# Autodesk Inventor assembly: Frame
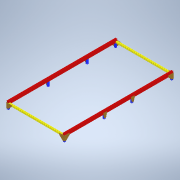
[picture p0: Inventor's stored thumbnail of the model, 180x180]
Saved by Autodesk Inventor 2022.2 (Build 262287010, 287A)
## iProperties
Created: 2022-03-31
Part Number: Frame
Document SubType Name: Assembly
Designer: Robert Nies
Author: Robert Nies
## Documents named in this file (6)
- C:\Users\rober\PycharmProjects\CNCRouter\Master Assembly\Frame.iam
- C:\Users\rober\PycharmProjects\CNCRouter\Master Assembly\Frame Long.ipt
- C:\Users\rober\PycharmProjects\CNCRouter\Master Assembly\Frame Short.ipt
- C:\Users\rober\PycharmProjects\CNCRouter\Master Assembly\Leg.ipt
- C:\Users\rober\PycharmProjects\CNCRouter\Stock Parts\Brackets\90 Deg 5 Hole Bracket.ipt
- C:\Users\rober\PycharmProjects\CNCRouter\Stock Parts\Brackets\Tee 4 Hole Bracket.ipt
## Components (26 placed, 5 different names)
1. Frame Short:2 — Mate:8, Flush:15, Flush:16, Flush:26, Flush:33, Flush:43, Flush:45, Flush:47
2. Frame Short:1 — Mate:3, Flush:5, Flush:6, Flush:13, Mate:7, Flush:14, Flush:20, Flush:39, Flush:41
3. Frame Long:1 — Flush:1, Flush:2, Mate:1, Mate:20, Flush:32, Mate:21, Flush:34, Mate:22, Flush:35, Mate:29, Flush:48
4. Frame Long:2 — Flush:1, Flush:2, Mate:1, Mate:3, Flush:5, Flush:6, Flush:17, Mate:9, Flush:18, Mate:19, Flush:31, Mate:23, Flush:36, Mate:25, Mate:26
5. Frame Long:3 — Flush:3, Flush:4, Mate:2, Mate:8, Flush:15, Flush:16, Flush:24, Mate:14, Mate:15, Mate:17, Flush:27, Flush:28, Flush:29, Mate:18, Mate:27, Mate:28, Flush:46
6. Frame Long:4 — Flush:3, Flush:4, Mate:2, Mate:6, Flush:11, Flush:12, Flush:13, Mate:7, Flush:14, Flush:19, Mate:11, Mate:12, Flush:23
7. Leg:8 — Mate:23, Flush:36, Mate:24
8. Leg:7 — Mate:21, Flush:33, Flush:34, Mate:30, Flush:50
9. Leg:6 — Mate:15, Mate:16, Flush:26, Flush:27, Flush:44
10. Leg:5 — Mate:10, Flush:19, Mate:11, Flush:25
11. Leg:4 — Mate:16, Mate:17, Flush:28, Flush:30
12. Leg:3 — Mate:22, Flush:35, Flush:38
13. Leg:2 — Flush:17, Mate:9, Flush:18, Mate:24, Flush:40
14. Leg:1 — Mate:6, Flush:11, Flush:12, Mate:10, Flush:21, Mate:13
15. 90 Deg 5 Hole Bracket:3 — Mate:25, Flush:39, Flush:40, Flush:42
16. 90 Deg 5 Hole Bracket:4 — Mate:26, Flush:41, Flush:42
17. 90 Deg 5 Hole Bracket:5 — Mate:27, Flush:43, Flush:44
18. 90 Deg 5 Hole Bracket:6 — Mate:28, Flush:45, Flush:46
19. 90 Deg 5 Hole Bracket:7 — Flush:47, Mate:29, Flush:48, Flush:49
20. 90 Deg 5 Hole Bracket:8 — Mate:30, Flush:49, Flush:50
21. Tee 4 Hole Bracket:2 — Flush:29, Mate:18, Flush:30
22. Tee 4 Hole Bracket:3 — Mate:19, Flush:31, Flush:37
23. Tee 4 Hole Bracket:4 — Mate:20, Flush:32, Flush:38
24. Tee 4 Hole Bracket:1 — Flush:24, Mate:14, Flush:25, Flush:37
25. 90 Deg 5 Hole Bracket:2 — Flush:22, Mate:13, Flush:23
26. 90 Deg 5 Hole Bracket:1 — Flush:20, Flush:21, Mate:12, Flush:22
## Relationships (74: Flush 46, Mate 28)
- Flush:1: Frame Long:1 ↔ Frame Long:2
- Flush:2: Frame Long:1 ↔ Frame Long:2
- Mate:1: Frame Long:1 ↔ Frame Long:2
- Flush:3: Frame Long:3 ↔ Frame Long:4
- Flush:4: Frame Long:3 ↔ Frame Long:4
- Mate:2: Frame Long:3 ↔ Frame Long:4
- Mate:3: Frame Short:1 ↔ Frame Long:2
- Flush:5: Frame Short:1 ↔ Frame Long:2
- Flush:6: Frame Short:1 ↔ Frame Long:2
- Mate:6: Frame Long:4 ↔ Leg:1
- Flush:11: Frame Long:4 ↔ Leg:1
- Flush:12: Frame Long:4 ↔ Leg:1
- Flush:13: Frame Short:1 ↔ Frame Long:4
- Mate:7: Frame Short:1 ↔ Frame Long:4
- Flush:14: Frame Short:1 ↔ Frame Long:4
- Mate:8: Frame Short:2 ↔ Frame Long:3
- Flush:15: Frame Short:2 ↔ Frame Long:3
- Flush:16: Frame Short:2 ↔ Frame Long:3
- Flush:17: Frame Long:2 ↔ Leg:2
- Mate:9: Frame Long:2 ↔ Leg:2
- Flush:18: Frame Long:2 ↔ Leg:2
- Mate:10 (889 mm): Leg:5 ↔ Leg:1
- Flush:19: Frame Long:4 ↔ Leg:5
- Mate:11: Frame Long:4 ↔ Leg:5
- Flush:20: Frame Short:1 ↔ 90 Deg 5 Hole Bracket:1
- Flush:21: Leg:1 ↔ 90 Deg 5 Hole Bracket:1
- Mate:12: Frame Long:4 ↔ 90 Deg 5 Hole Bracket:1
- Flush:22: 90 Deg 5 Hole Bracket:2 ↔ 90 Deg 5 Hole Bracket:1
- Mate:13: Leg:1 ↔ 90 Deg 5 Hole Bracket:2
- Flush:23: Frame Long:4 ↔ 90 Deg 5 Hole Bracket:2
- Flush:24 (38.1 mm): Frame Long:3 ↔ Tee 4 Hole Bracket:1
- Mate:14: Frame Long:3 ↔ Tee 4 Hole Bracket:1
- Flush:25 (19.05 mm): Leg:5 ↔ Tee 4 Hole Bracket:1
- Mate:15: Frame Long:3 ↔ Leg:6
- Mate:16 (889 mm): Leg:6 ↔ Leg:4
- Mate:17: Frame Long:3 ↔ Leg:4
- Flush:26: Frame Short:2 ↔ Leg:6
- Flush:27: Frame Long:3 ↔ Leg:6
- Flush:28: Frame Long:3 ↔ Leg:4
- Flush:29 (38.1 mm): Frame Long:3 ↔ Tee 4 Hole Bracket:2
- Mate:18: Frame Long:3 ↔ Tee 4 Hole Bracket:2
- Flush:30 (-19.05 mm): Leg:4 ↔ Tee 4 Hole Bracket:2
- Mate:19: Frame Long:2 ↔ Tee 4 Hole Bracket:3
- Mate:20: Frame Long:1 ↔ Tee 4 Hole Bracket:4
- Flush:31 (38.1 mm): Frame Long:2 ↔ Tee 4 Hole Bracket:3
- Flush:32 (38.1 mm): Frame Long:1 ↔ Tee 4 Hole Bracket:4
- Mate:21: Frame Long:1 ↔ Leg:7
- Flush:33: Frame Short:2 ↔ Leg:7
- Flush:34: Frame Long:1 ↔ Leg:7
- Mate:22: Frame Long:1 ↔ Leg:3
- Flush:35: Frame Long:1 ↔ Leg:3
- Mate:23: Frame Long:2 ↔ Leg:8
- Flush:36: Frame Long:2 ↔ Leg:8
- Mate:24 (889 mm): Leg:8 ↔ Leg:2
- Flush:37: Tee 4 Hole Bracket:3 ↔ Tee 4 Hole Bracket:1
- Flush:38 (19.05 mm): Leg:3 ↔ Tee 4 Hole Bracket:4
- Mate:25: Frame Long:2 ↔ 90 Deg 5 Hole Bracket:3
- Flush:39: Frame Short:1 ↔ 90 Deg 5 Hole Bracket:3
- Flush:40: Leg:2 ↔ 90 Deg 5 Hole Bracket:3
- Mate:26: Frame Long:2 ↔ 90 Deg 5 Hole Bracket:4
- Flush:41: Frame Short:1 ↔ 90 Deg 5 Hole Bracket:4
- Flush:42: 90 Deg 5 Hole Bracket:3 ↔ 90 Deg 5 Hole Bracket:4
- Mate:27: Frame Long:3 ↔ 90 Deg 5 Hole Bracket:5
- Flush:43: Frame Short:2 ↔ 90 Deg 5 Hole Bracket:5
- Flush:44: Leg:6 ↔ 90 Deg 5 Hole Bracket:5
- Mate:28: Frame Long:3 ↔ 90 Deg 5 Hole Bracket:6
- Flush:45: Frame Short:2 ↔ 90 Deg 5 Hole Bracket:6
- Flush:46: Frame Long:3 ↔ 90 Deg 5 Hole Bracket:6
- Flush:47: Frame Short:2 ↔ 90 Deg 5 Hole Bracket:7
- Mate:29: Frame Long:1 ↔ 90 Deg 5 Hole Bracket:7
- Flush:48: Frame Long:1 ↔ 90 Deg 5 Hole Bracket:7
- Mate:30: Leg:7 ↔ 90 Deg 5 Hole Bracket:8
- Flush:49: 90 Deg 5 Hole Bracket:7 ↔ 90 Deg 5 Hole Bracket:8
- Flush:50: Leg:7 ↔ 90 Deg 5 Hole Bracket:8
## Named parameters: d3_d0 = 0 mm, d4_d1 = 0 mm, d5_d2 = 0 mm
